# Autodesk Inventor assembly: Squiggle_Motor_Base
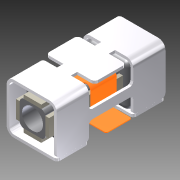
[picture p0: Inventor's stored thumbnail of the model, 180x180]
Saved by Autodesk Inventor 2011 SP2 (Build 150309200, 309)
## iProperties
Created: 2011-09-20
Part Number: Squiggle_Motor_Base
Document SubType Name: Assembly
Designer: sungwook
Author: sungwook
## Documents named in this file (7)
- C:\Users\sungwook\Documents\Inventor\Micron18_Tension_Merge_Test\Motor_Unit\MU_SQ_Motor_Base.iam
- C:\Users\sungwook\Documents\Inventor\Micron18_Tension_Merge_Test\Motor_Unit\SQ_Motors\Frame.ipt
- C:\Users\sungwook\Documents\Inventor\Micron18_Tension_Merge_Test\Motor_Unit\SQ_Motors\PZT_Guide.ipt
- C:\Users\sungwook\Documents\Inventor\Micron18_Tension_Merge_Test\Motor_Unit\SQ_Motors\Piezoelectric_Element.ipt
- C:\Users\sungwook\Documents\Inventor\Micron18_Tension_Merge_Test\Motor_Unit\SQ_Motors\FPCB.ipt
- C:\Users\sungwook\Documents\Inventor\Micron18_Tension_Merge_Test\Motor_Unit\SQ_Motors\Frame_Support2.ipt
- C:\Users\sungwook\Documents\Inventor\Micron18_Tension_Merge_Test\Motor_Unit\SQ_Motors\Frame_Support2_MIR1.ipt
## Components (9 placed, 6 different names)
1. Frame:1 — Mate:11, Mate:12, Flush:3, Mate:13, Mate:14, Flush:4
2. PZT_Guide:1 — Mate:15, Mate:16, Mate:17
3. FPCB:1 — Mate:22, Mate:24, Flush:5
4. Frame_Support2:1 — Mate:11, Mate:12, Flush:3
5. Frame_Support2_MIR1:1 — Mate:13, Mate:14, Flush:4, Mate:15, Mate:16, Mate:19, Mate:21
6. Piezoelectric_Element:1 — Mate:19, Mate:20, Mate:21
7. Piezoelectric_Element:2
8. Piezoelectric_Element:3 — Mate:24
9. Piezoelectric_Element:4 — Mate:22
## Component patterns: (4 elements, first: Piezoelectric_Element:1)
## Relationships (15: Mate 12, Flush 3)
- Mate:11: Frame:1 ↔ Frame_Support2:1
- Mate:12: Frame:1 ↔ Frame_Support2:1
- Flush:3 (-0.727 mm): Frame:1 ↔ Frame_Support2:1
- Mate:13: Frame:1 ↔ Frame_Support2_MIR1:1
- Mate:14: Frame:1 ↔ Frame_Support2_MIR1:1
- Flush:4 (0.727 mm): Frame:1 ↔ Frame_Support2_MIR1:1
- Mate:15: PZT_Guide:1 ↔ Frame_Support2_MIR1:1
- Mate:16: PZT_Guide:1 ↔ Frame_Support2_MIR1:1
- Mate:17: PZT_Guide:1
- Mate:19: Frame_Support2_MIR1:1 ↔ Piezoelectric_Element:1
- Mate:20: Piezoelectric_Element:1
- Mate:21: Frame_Support2_MIR1:1 ↔ Piezoelectric_Element:1
- Mate:22: FPCB:1 ↔ Piezoelectric_Element:4
- Mate:24: FPCB:1 ↔ Piezoelectric_Element:3
- Flush:5: FPCB:1
